# Autodesk Inventor assembly: Ensemble1
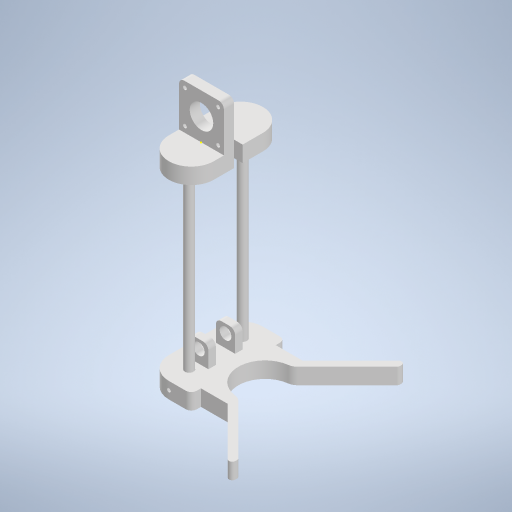
[picture p0: Inventor's stored thumbnail of the model, 512x512]
Saved by Autodesk Inventor 2024.1 (Build 281209000, 209)
## iProperties
Created: 2024-04-06
Part Number: Ensemble1
Document SubType Name: Assembly
Designer: chass
Author: chass
## Documents named in this file (4)
- C:\Users\chass\Desktop\Actionneur_robot_cdr\Ensemble1.iam
- C:\Users\chass\Desktop\Actionneur_robot_cdr\bas.ipt
- C:\Users\chass\Desktop\Actionneur_robot_cdr\Tige_rail.ipt
- C:\Users\chass\Desktop\Actionneur_robot_cdr\tete.ipt
## Components (4 placed, 3 different names)
1. bas:1 — Placage:1, Placage:2
2. Tige_rail:1 — Placage:2, Placage:4, Placage:6
3. Tige_rail:2 — Placage:1, Placage:3, Placage:5
4. tete:1 — Placage:3, Placage:4, Placage:5, Placage:6
## Relationships (6: Mate 6)
- Placage:1 [Mate]: bas:1 ↔ Tige_rail:2
- Placage:2 [Mate]: bas:1 ↔ Tige_rail:1
- Placage:3 [Mate]: Tige_rail:2 ↔ tete:1
- Placage:4 [Mate]: Tige_rail:1 ↔ tete:1
- Placage:5 [Mate]: Tige_rail:2 ↔ tete:1
- Placage:6 [Mate]: Tige_rail:1 ↔ tete:1
